# Autodesk Inventor assembly: Assembled Mudbox Claw R
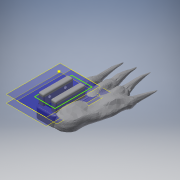
[picture p0: Inventor's stored thumbnail of the model, 180x180]
Saved by Autodesk Inventor 2019 (Build 230136000, 136)
## iProperties
Created: 2019-06-12
Part Number: Assembled Mudbox Claw R
Document SubType Name: Assembly
Designer: Cole
Author: Cole
## Documents named in this file (3)
- G:\My Drive\Clubs\MTHS TSA\Animatronics 2019\Glyptodon\Glyptodon Work\Arms\Assembled Mudbox Claw R.iam
- G:\My Drive\Clubs\MTHS TSA\Animatronics 2019\Glyptodon\Glyptodon Work\Arms\Scaled Foot R.ipt
- C:\Users\Cole\Documents\temp.ipt
## Components (2 placed, 2 different names)
1. Scaled Foot R:1 — Flush:1
2. temp:1 — Flush:1
## Relationships (1: Flush 1)
- Flush:1: Scaled Foot R:1 ↔ temp:1
